# Autodesk Inventor assembly: full door assembly
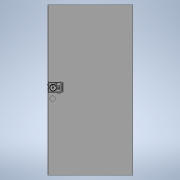
[picture p0: Inventor's stored thumbnail of the model, 180x180]
Saved by Autodesk Inventor 2022 (Build 260153000, 153)
## iProperties
Created: 2022-06-16
Part Number: full door assembly
Document SubType Name: Assembly
Designer: alecw
Author: alecw
## Documents named in this file (4)
- C:\aw_gd\Coding and Projects\smart home\smart-deadbolt\3D Modelling\full door assembly.iam
- C:\aw_gd\Coding and Projects\smart home\smart-deadbolt\3D Modelling\door.ipt
- C:\aw_gd\Coding and Projects\smart home\smart-deadbolt\3D Modelling\deadbolt arm.ipt
- C:\aw_gd\Coding and Projects\smart home\smart-deadbolt\3D Modelling\full deadbolt controller enclosure assembly.iam
## Components (3 placed, 3 different names)
1. door:1 — Cylindrical:3, Mate:2, Mate:4, Mate:5, Mate:6, Mate:7, Mate:8, Mate:9, Mate:10
2. deadbolt arm:1 — Cylindrical:3, Mate:6, Mate:8
3. full deadbolt controller enclosure assembly:1 [sub-assembly] — Mate:4, Mate:5, Mate:9, Mate:10
## Relationships (9: Mate 8, CylindricalJoint 1)
- Cylindrical:3: door:1 ↔ deadbolt arm:1
- Mate:2: door:1
- Mate:4: door:1 ↔ full deadbolt controller enclosure assembly:1
- Mate:5: door:1 ↔ full deadbolt controller enclosure assembly:1
- Mate:6: door:1 ↔ deadbolt arm:1
- Mate:7: door:1
- Mate:8: door:1 ↔ deadbolt arm:1
- Mate:9: door:1 ↔ full deadbolt controller enclosure assembly:1
- Mate:10: door:1 ↔ full deadbolt controller enclosure assembly:1
